# Autodesk Inventor assembly: 1 door
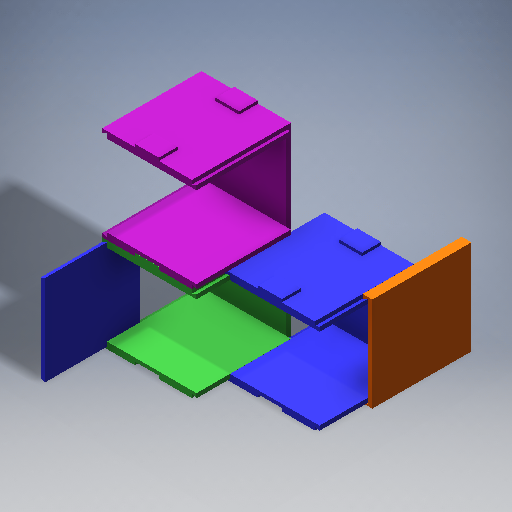
[picture p0: Inventor's stored thumbnail of the model, 512x512]
Saved by Autodesk Inventor 2025.2 (Build 292293000, 293)
## iProperties
Created: 2025-02-23
Part Number: 1 door
Document SubType Name: Assembly
Designer: Alex
Author: Alex
## Documents named in this file (4)
- C:\Shared\alex-bartella-schoolwork\4b03\dr2\1 door.iam
- C:\Shared\alex-bartella-schoolwork\4b03\dr2\main - 1 door.ipt
- C:\Shared\alex-bartella-schoolwork\4b03\dr2\door2.ipt
- C:\Shared\alex-bartella-schoolwork\4b03\dr2\door3.ipt
## Components (8 placed, 3 different names)
1. main - 1 door:1 — Flush:1, Mate:1, Flush:3, Flush:4, Flush:5, Mate:2, Mate:5, Flush:7, Mate:10, Flush:11, Flush:12
2. main - 1 door:2 — Flush:1, Mate:1, Flush:3, Flush:6
3. door2:1 — Flush:4, Flush:5, Mate:2
4. door3:1 — Flush:6
5. main - 1 door:3 — Mate:3, Mate:4, Flush:8, Mate:6, Flush:9, Mate:7, Mate:8, Mate:9, Flush:10
6. door2:2 — Flush:8, Mate:6, Flush:9
7. door3:2 — Mate:8, Mate:9, Flush:10
8. main - 1 door:4 — Mate:10, Flush:11, Flush:12
## Relationships (21: Flush 11, Mate 10)
- Flush:1: main - 1 door:1 ↔ main - 1 door:2
- Mate:1 (0.1 mm): main - 1 door:1 ↔ main - 1 door:2
- Flush:3: main - 1 door:1 ↔ main - 1 door:2
- Flush:4: main - 1 door:1 ↔ door2:1
- Flush:5 (0.1 mm): main - 1 door:1 ↔ door2:1
- Mate:2 (0.1 mm): main - 1 door:1 ↔ door2:1
- Flush:6: main - 1 door:2 ↔ door3:1
- Mate:3 (180 mm): main - 1 door:3
- Mate:4: main - 1 door:3
- Mate:5: main - 1 door:1
- Flush:7: main - 1 door:1
- Flush:8: main - 1 door:3 ↔ door2:2
- Mate:6 (0.1 mm): main - 1 door:3 ↔ door2:2
- Flush:9: main - 1 door:3 ↔ door2:2
- Mate:7: main - 1 door:3
- Mate:8: main - 1 door:3 ↔ door3:2
- Mate:9 (0.1 mm): main - 1 door:3 ↔ door3:2
- Flush:10: main - 1 door:3 ↔ door3:2
- Mate:10: main - 1 door:1 ↔ main - 1 door:4
- Flush:11: main - 1 door:1 ↔ main - 1 door:4
- Flush:12: main - 1 door:1 ↔ main - 1 door:4
